# Autodesk Inventor assembly: screw_left
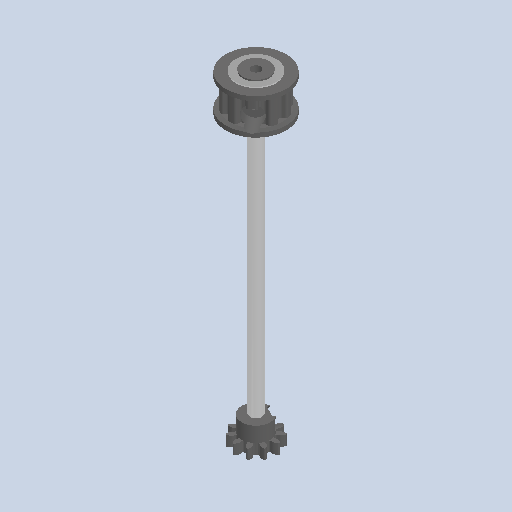
[picture p0: Inventor's stored thumbnail of the model, 512x512]
Saved by Autodesk Inventor 2024.1 (Build 281209000, 209)
## iProperties
Created: 2025-01-17
Part Number: screw_left
Document SubType Name: Assembly
Designer: hibik
Author: hibik
## Documents named in this file (7)
- C:\Users\hibik\Documents\Robomech\RESCUE\ORCA\hard\fork\left\screw_left.iam
- C:\Users\hibik\Documents\Robomech\RESCUE\ORCA\hard\fork\left\screw_screw_left.ipt
- C:\Users\hibik\Documents\Robomech\RESCUE\ORCA\hard\fork\left\bearing_6_10_3_left.ipt
- C:\Users\hibik\Documents\Robomech\RESCUE\ORCA\hard\fork\left\screw_bearing_setter_left.ipt
- C:\Users\hibik\Documents\Robomech\RESCUE\ORCA\hard\fork\left\bearing_3_6_2.5_noscrew_left.ipt
- C:\Users\hibik\Documents\Robomech\RESCUE\ORCA\hard\fork\left\screw_gear_under_12_left.ipt
- C:\Users\hibik\Documents\Robomech\RESCUE\ORCA\hard\fork\left\screw_gear_upper_left.ipt
## Components (6 placed, 6 different names)
1. screw_screw_left:1 — 挿入:9, 挿入:11
2. bearing_6_10_3_left:1 — 挿入:7, 挿入:8
3. screw_bearing_setter_left:1 — 挿入:9, 挿入:7
4. bearing_3_6_2.5_noscrew_left:1 — 挿入:11, 挿入:10
5. screw_gear_under_12_left:1 — 挿入:10
6. screw_gear_upper_left:1 — 挿入:8
## Relationships (5: Insert 5)
- 挿入:9 [Insert]: screw_screw_left:1 ↔ screw_bearing_setter_left:1
- 挿入:7 [Insert]: bearing_6_10_3_left:1 ↔ screw_bearing_setter_left:1
- 挿入:11 [Insert] (1 mm): screw_screw_left:1 ↔ bearing_3_6_2.5_noscrew_left:1
- 挿入:10 [Insert]: bearing_3_6_2.5_noscrew_left:1 ↔ screw_gear_under_12_left:1
- 挿入:8 [Insert]: bearing_6_10_3_left:1 ↔ screw_gear_upper_left:1
